# Autodesk Inventor assembly: Estacion_Corte
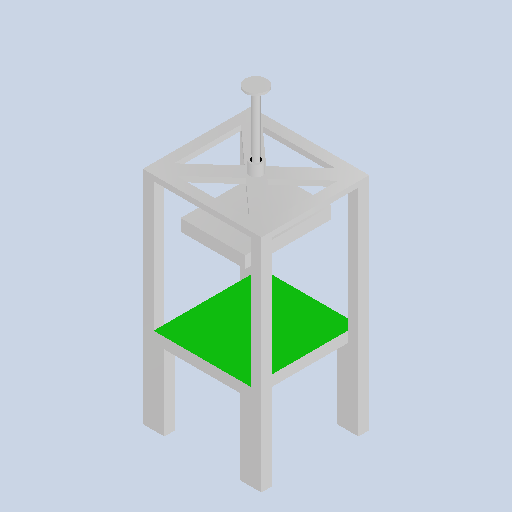
[picture p0: Inventor's stored thumbnail of the model, 512x512]
Saved by Autodesk Inventor 2025.2 (Build 292293000, 293)
## iProperties
Created: 2025-02-05
Part Number: Estacion_Corte
Document SubType Name: Assembly
Designer: Proyectos
Author: Proyectos
## Documents named in this file (3)
- C:\Users\hmont\OneDrive\Desktop\2024-2\Automatizacion de Procesos de Manufactura\Modelado\Cortadora\Estacion_Corte.iam
- C:\Users\hmont\OneDrive\Desktop\2024-2\Automatizacion de Procesos de Manufactura\Modelado\Cortadora\Corte.ipt
- C:\Users\hmont\OneDrive\Desktop\2024-2\Automatizacion de Procesos de Manufactura\Modelado\Cortadora\Soporte_Corte.ipt
## Components (2 placed, 2 different names)
1. Corte:1 — Coincidencia:1
2. Soporte_Corte:1 — Coincidencia:1
## Relationships (1: Mate 1)
- Coincidencia:1 [Mate]: Corte:1 ↔ Soporte_Corte:1
